# Autodesk Inventor assembly: 足全体
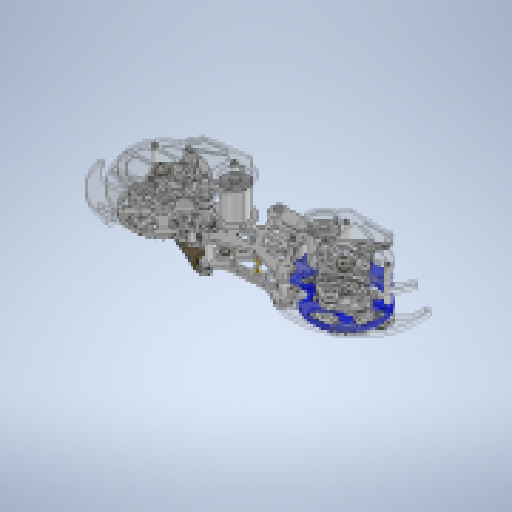
[picture p0: Inventor's stored thumbnail of the model, 512x512]
Saved by Autodesk Inventor 2023 (Build 270158000, 158)
## iProperties
Created: 2022-01-30
Part Number: 足全体
Document SubType Name: Assembly
Designer: acps
Author: acps
## Documents named in this file (11)
- C:\Users\muzho\Documents\srdc\srdc_2\脚\足全体.iam
- C:\Users\muzho\Documents\srdc\srdc_2\脚\足ユニット.iam
- C:\Users\muzho\Documents\srdc\srdc_2\スペーサ\l23.ipt
- C:\Users\muzho\Documents\srdc\srdc_2\タミヤダンパー1.iam
- C:\Users\muzho\Documents\srdc\srdc_2\スペーサ\l10.ipt
- C:\Users\muzho\Documents\srdc\srdc_2\脚\中間ユニット内_MIR1.ipt
- C:\Users\muzho\Documents\srdc\srdc_2\脚\中間ユニット外(shin).ipt
- C:\Users\muzho\Documents\srdc\srdc_2\スペーサ\l7.ipt
- C:\Users\muzho\Documents\srdc\srdc_2\脚\足ユニット_MIR.iam
- C:\Users\muzho\Documents\srdc\srdc_2\脚\ミラー\l10_MIR.ipt
- C:\Users\muzho\Documents\srdc\srdc_2\脚\ミラー\l7_MIR.ipt
## Components (18 placed, 10 different names)
1. 足ユニット:1 [sub-assembly] — 挿入:17, 挿入:23
2. l23:1 — 挿入:33
3. l23:2 — 挿入:32
4. l23:3
5. l23:4 — 挿入:16
6. l23:5 — 挿入:28
7. l23:6 — 挿入:19, 挿入:21
8. l23:7 — 挿入:22
9. l23:8 — 挿入:20, メイト:5
10. タミヤダンパー1:1 [sub-assembly] — 挿入:24
11. l10:1 — 挿入:23, 挿入:24
12. 中間ユニット内_MIR1:1 — 挿入:16, 挿入:17, 挿入:19, 挿入:20, 挿入:22, 挿入:25, 挿入:28, 挿入:31, 挿入:32, 挿入:33
13. 中間ユニット外(shin):1 — メイト:5, 挿入:21
14. l7:1 — 挿入:25
15. 足ユニット_MIR:1 [sub-assembly] — 挿入:34
16. l10_MIR:1 — メイト:8, 挿入:30, 挿入:34
17. l7_MIR:1 — 挿入:31
18. タミヤダンパー1:2 [sub-assembly] — メイト:8, 挿入:30
## Relationships (17: Insert 15, Mate 2)
- 挿入:16 [Insert]: l23:4 ↔ 中間ユニット内_MIR1:1
- 挿入:17 [Insert]: 足ユニット:1 ↔ 中間ユニット内_MIR1:1
- 挿入:19 [Insert]: l23:6 ↔ 中間ユニット内_MIR1:1
- 挿入:20 [Insert]: l23:8 ↔ 中間ユニット内_MIR1:1
- メイト:5 [Mate]: l23:8 ↔ 中間ユニット外(shin):1
- 挿入:21 [Insert]: l23:6 ↔ 中間ユニット外(shin):1
- 挿入:22 [Insert]: l23:7 ↔ 中間ユニット内_MIR1:1
- 挿入:23 [Insert]: 足ユニット:1 ↔ l10:1
- 挿入:24 [Insert]: タミヤダンパー1:1 ↔ l10:1
- 挿入:25 [Insert]: 中間ユニット内_MIR1:1 ↔ l7:1
- 挿入:28 [Insert]: l23:5 ↔ 中間ユニット内_MIR1:1
- メイト:8 [Mate]: l10_MIR:1 ↔ タミヤダンパー1:2
- 挿入:30 [Insert]: l10_MIR:1 ↔ タミヤダンパー1:2
- 挿入:31 [Insert]: 中間ユニット内_MIR1:1 ↔ l7_MIR:1
- 挿入:32 [Insert]: l23:2 ↔ 中間ユニット内_MIR1:1
- 挿入:33 [Insert]: l23:1 ↔ 中間ユニット内_MIR1:1
- 挿入:34 [Insert]: 足ユニット_MIR:1 ↔ l10_MIR:1
